# Autodesk Inventor assembly: BackLink
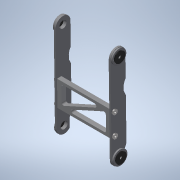
[picture p0: Inventor's stored thumbnail of the model, 180x180]
Saved by Autodesk Inventor 2020.4 (Build 244396000, 396)
## iProperties
Created: 2016-08-23
Part Number: BackLink
Material: 一般
Document SubType Name: Assembly
Designer: hiro
Mass: 27.0677 g
Surface Area: 148.123 cm^2
Volume: 12.1706 cm^3
Density: 2.22402 g/cm^3
Author: hiro
## Documents named in this file (6)
- C:\Users\Masato\Documents\Inventor\CIT Brains_Inventor\OpenPlatform_ver3_0\LowerBody\Link\BackLink.iam
- C:\Users\Masato\Documents\Inventor\CIT Brains_Inventor\OpenPlatform_ver3_0\LowerBody\Link\Link_back_side_frame.ipt
- C:\Users\Masato\Documents\Inventor\CIT Brains_Inventor\OpenPlatform_ver3_0\LowerBody\Link\Link_back_diagonal.ipt
- C:\Users\Masato\Documents\Inventor\CIT Brains_Inventor\OpenPlatform_ver3_0\Ready_Made\UUW-0312-10BH.ipt
- C:\Users\Masato\Documents\Inventor\CIT Brains_Inventor\OpenPlatform_ver3_0\Ready_Made\LFW-0815.ipt
- C:\Users\Masato\Documents\Inventor\CIT Brains_Inventor\OpenPlatform_ver3_0\Ready_Made\Screw\M3-6.ipt
## Components (15 placed, 5 different names)
1. Link_back_side_frame:1 — 挿入:17, 挿入:21, 挿入:22, 挿入:31, 挿入:33, 挿入:34
2. Link_back_side_frame:2 — 挿入:18, 挿入:23, 挿入:24, 挿入:32, 挿入:35, 挿入:36
3. UUW-0312-10BH:1 — 挿入:30
4. UUW-0312-10BH:2 — 挿入:29
5. UUW-0312-10BH:3 — 挿入:20
6. UUW-0312-10BH:4 — 挿入:19
7. LFW-0815:1 — 挿入:18, 挿入:20
8. LFW-0815:2 — 挿入:17, 挿入:19
9. Link_back_diagonal:1 — 挿入:21, 挿入:22, 挿入:23, 挿入:24
10. LFW-0815:3 — 挿入:29, 挿入:32
11. LFW-0815:4 — 挿入:30, 挿入:31
12. M3-6:1 — 挿入:36
13. M3-6:2 — 挿入:35
14. M3-6:3 — 挿入:34
15. M3-6:4 — 挿入:33
## Relationships (16: Insert 16)
- 挿入:17 [Insert]: Link_back_side_frame:1 ↔ LFW-0815:2
- 挿入:18 [Insert]: Link_back_side_frame:2 ↔ LFW-0815:1
- 挿入:19 [Insert]: UUW-0312-10BH:4 ↔ LFW-0815:2
- 挿入:20 [Insert]: UUW-0312-10BH:3 ↔ LFW-0815:1
- 挿入:21 [Insert]: Link_back_side_frame:1 ↔ Link_back_diagonal:1
- 挿入:22 [Insert]: Link_back_side_frame:1 ↔ Link_back_diagonal:1
- 挿入:23 [Insert]: Link_back_side_frame:2 ↔ Link_back_diagonal:1
- 挿入:24 [Insert]: Link_back_side_frame:2 ↔ Link_back_diagonal:1
- 挿入:29 [Insert]: UUW-0312-10BH:2 ↔ LFW-0815:3
- 挿入:30 [Insert]: UUW-0312-10BH:1 ↔ LFW-0815:4
- 挿入:31 [Insert]: Link_back_side_frame:1 ↔ LFW-0815:4
- 挿入:32 [Insert]: Link_back_side_frame:2 ↔ LFW-0815:3
- 挿入:33 [Insert]: Link_back_side_frame:1 ↔ M3-6:4
- 挿入:34 [Insert]: Link_back_side_frame:1 ↔ M3-6:3
- 挿入:35 [Insert]: Link_back_side_frame:2 ↔ M3-6:2
- 挿入:36 [Insert]: Link_back_side_frame:2 ↔ M3-6:1
